# Autodesk Inventor assembly: Assembly of Parts
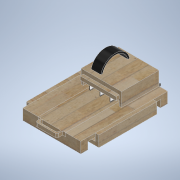
[picture p0: Inventor's stored thumbnail of the model, 180x180]
Saved by Autodesk Inventor 2022 (Build 260153000, 153)
## iProperties
Created: 2022-04-15
Part Number: Assembly of Parts
Document SubType Name: Assembly
Designer: mpate
Author: mpate
## Documents named in this file (11)
- C:\Users\mpate\Desktop\Thurs-41_P4_CAD_Files\Assembly of Parts.iam
- C:\Users\mpate\Desktop\Thurs-41_P4_CAD_Files\Cutting Board without Cutout.ipt
- C:\Users\mpate\Desktop\Thurs-41_P4_CAD_Files\Cutting Board Cutout.ipt
- C:\Users\mpate\Desktop\Thurs-41_P4_CAD_Files\Hinge Bottom.ipt
- C:\Users\mpate\Desktop\Thurs-41_P4_CAD_Files\Drawer.ipt
- C:\Users\mpate\Desktop\Thurs-41_P4_CAD_Files\Slicer.ipt
- C:\Users\mpate\Desktop\Thurs-41_P4_CAD_Files\Hinge Top.ipt
- C:\Users\mpate\Desktop\Thurs-41_P4_CAD_Files\Blade Insert.ipt
- C:\Users\mpate\Desktop\Thurs-41_P4_CAD_Files\Hinge Pin.ipt
- C:\Users\mpate\Desktop\Thurs-41_P4_CAD_Files\Blade.ipt
- C:\Users\mpate\Desktop\Thurs-41_P4_CAD_Files\Slicer Strap.ipt
## Components (15 placed, 10 different names)
1. Cutting Board without Cutout:1 — Mate:1, Mate:2, Mate:3, Flush:1, Mate:4, Mate:5, Mate:6, Mate:7, Mate:8, Mate:9, Mate:10, Mate:11, Angle:1
2. Cutting Board Cutout:1 — Mate:1, Mate:2, Mate:3
3. Hinge Bottom:1 — Mate:6, Mate:7, Mate:8, Insert:2
4. Hinge Bottom:2 — Mate:9, Mate:10, Mate:11, Mate:28, Mate:29, Insert:1
5. Drawer:1 — Flush:1, Mate:4, Mate:5
6. Slicer:1 — Mate:13, Mate:14, Mate:15, Mate:16, Mate:17, Mate:18, Mate:19, Flush:2, Mate:20, Mate:25, Mate:26, Mate:27, Angle:1
7. Hinge Top:1 — Mate:13, Mate:14, Mate:15
8. Hinge Top:2 — Mate:16, Mate:17, Mate:18, Mate:28, Mate:29
9. Blade Insert:1 — Mate:21, Mate:22, Mate:23, Flush:3, Flush:4, Flush:5, Flush:6, Flush:7, Mate:25, Mate:26, Mate:27
10. Hinge Pin:1 — Insert:1
11. Hinge Pin:2 — Insert:2
12. Blade:1 — Mate:21, Flush:4, Mate:24
13. Blade:2 — Mate:22, Flush:3, Flush:6, Mate:24
14. Blade:3 — Mate:23, Flush:5, Flush:7
15. Slicer Strap:1 — Mate:19, Flush:2, Mate:20
## Relationships (38: Mate 28, Flush 7, Insert 2, Angle 1)
- Mate:1: Cutting Board without Cutout:1 ↔ Cutting Board Cutout:1
- Mate:2: Cutting Board without Cutout:1 ↔ Cutting Board Cutout:1
- Mate:3: Cutting Board without Cutout:1 ↔ Cutting Board Cutout:1
- Flush:1: Cutting Board without Cutout:1 ↔ Drawer:1
- Mate:4 (38.1 mm): Cutting Board without Cutout:1 ↔ Drawer:1
- Mate:5: Cutting Board without Cutout:1 ↔ Drawer:1
- Mate:6: Cutting Board without Cutout:1 ↔ Hinge Bottom:1
- Mate:7: Cutting Board without Cutout:1 ↔ Hinge Bottom:1
- Mate:8: Cutting Board without Cutout:1 ↔ Hinge Bottom:1
- Mate:9: Cutting Board without Cutout:1 ↔ Hinge Bottom:2
- Mate:10: Cutting Board without Cutout:1 ↔ Hinge Bottom:2
- Mate:11: Cutting Board without Cutout:1 ↔ Hinge Bottom:2
- Mate:13: Slicer:1 ↔ Hinge Top:1
- Mate:14: Slicer:1 ↔ Hinge Top:1
- Mate:15: Slicer:1 ↔ Hinge Top:1
- Mate:16: Slicer:1 ↔ Hinge Top:2
- Mate:17: Slicer:1 ↔ Hinge Top:2
- Mate:18: Slicer:1 ↔ Hinge Top:2
- Mate:19: Slicer:1 ↔ Slicer Strap:1
- Flush:2 (-30 mm): Slicer:1 ↔ Slicer Strap:1
- Mate:20 (-22.925 mm): Slicer:1 ↔ Slicer Strap:1
- Mate:21: Blade Insert:1 ↔ Blade:1
- Mate:22: Blade Insert:1 ↔ Blade:2
- Mate:23: Blade Insert:1 ↔ Blade:3
- Flush:3 (-9.4565 mm): Blade Insert:1 ↔ Blade:2
- Flush:4 (-9.4565 mm): Blade Insert:1 ↔ Blade:1
- Flush:5 (-9.4565 mm): Blade Insert:1 ↔ Blade:3
- Flush:6 (-40 mm): Blade Insert:1 ↔ Blade:2
- Flush:7 (-40 mm): Blade Insert:1 ↔ Blade:3
- Mate:24 (51.4565 mm): Blade:1 ↔ Blade:2
- Mate:25: Slicer:1 ↔ Blade Insert:1
- Mate:26: Slicer:1 ↔ Blade Insert:1
- Mate:27: Slicer:1 ↔ Blade Insert:1
- Mate:28: Hinge Bottom:2 ↔ Hinge Top:2
- Mate:29: Hinge Bottom:2 ↔ Hinge Top:2
- Insert:1: Hinge Bottom:2 ↔ Hinge Pin:1
- Insert:2: Hinge Bottom:1 ↔ Hinge Pin:2
- Angle:1 (0 deg): Cutting Board without Cutout:1 ↔ Slicer:1
